# Autodesk Inventor assembly: asPrototypedBallRamp_MIR
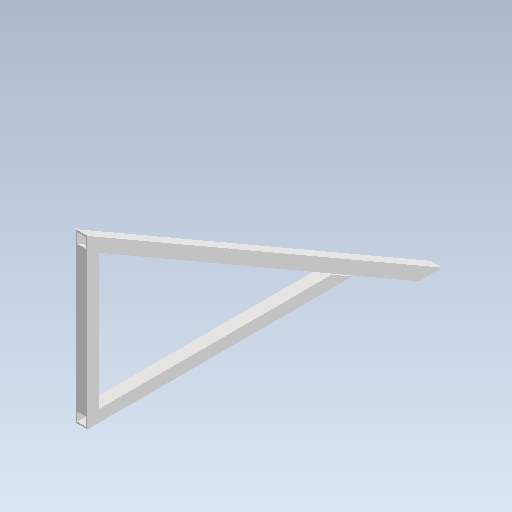
[picture p0: Inventor's stored thumbnail of the model, 512x512]
Saved by Autodesk Inventor 2020.2 (Build 242310000, 310)
## iProperties
Created: 2020-01-19
Part Number: asPrototypedBallRamp_MIR
Document SubType Name: Assembly
Designer: robst
Author: robst
## Documents named in this file (4)
- C:\git\CAD-Development\robSteele\2020LongRobotBase\asPrototypedBallRamp_MIR.iam
- C:\git\CAD-Development\robSteele\2020BallTriggerMechanism\baseAluminumExtrusion_MIR.ipt
- C:\git\CAD-Development\robSteele\2020LongRobotBase\sideAluminumExtrusion_MIR.ipt
- C:\git\CAD-Development\robSteele\2020LongRobotBase\hypotAluminumExtrusion_MIR.ipt
## Components (3 placed, 3 different names)
1. baseAluminumExtrusion_MIR:1 — Flush:2, Flush:1, Mate:1
2. sideAluminumExtrusion_MIR:1 — Flush:2, Flush:1, Mate:1, Mate:3, Flush:3, Mate:2
3. hypotAluminumExtrusion_MIR:1 — Mate:3, Flush:3, Mate:2
## Relationships (6: Flush 3, Mate 3)
- Flush:2: baseAluminumExtrusion_MIR:1 ↔ sideAluminumExtrusion_MIR:1
- Flush:1: baseAluminumExtrusion_MIR:1 ↔ sideAluminumExtrusion_MIR:1
- Mate:1: baseAluminumExtrusion_MIR:1 ↔ sideAluminumExtrusion_MIR:1
- Mate:3: sideAluminumExtrusion_MIR:1 ↔ hypotAluminumExtrusion_MIR:1
- Flush:3: sideAluminumExtrusion_MIR:1 ↔ hypotAluminumExtrusion_MIR:1
- Mate:2: sideAluminumExtrusion_MIR:1 ↔ hypotAluminumExtrusion_MIR:1
